# Autodesk Inventor assembly: zlozenie_wszystko
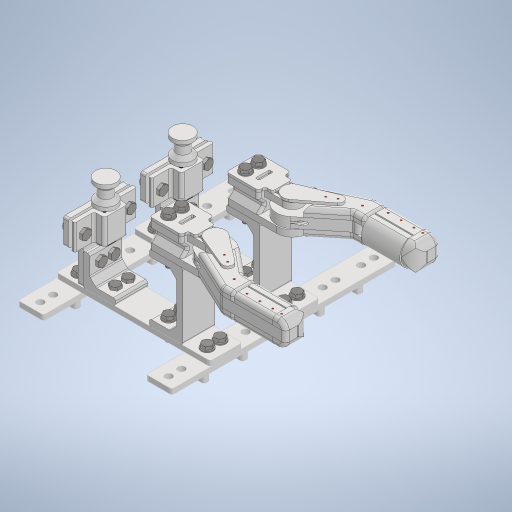
[picture p0: Inventor's stored thumbnail of the model, 512x512]
Saved by Autodesk Inventor 2024.2 (Build 282272000, 272)
## iProperties
Created: 2024-01-20
Part Number: zlozenie_wszystko
Document SubType Name: Assembly
Designer: Konrad
Author: Konrad
## Documents named in this file (9)
- D:\Inventor\magisterka\prototyp_2\zlozenie_wszystko.iam
- D:\Inventor\magisterka\prototyp_2\zlozenie_palec_lewy.iam
- D:\Inventor\magisterka\prototyp_2\zlozenie_palec_prawy.iam
- D:\Inventor\magisterka\prototyp_2\zlozenie_ramka.iam
- C:\Users\Konrad\Documents\Inventor\Content Center Files\R2024\pl-PL\DIN 125-1  A\DIN 125 - A 4,3.ipt
- C:\Users\Konrad\Documents\Inventor\Content Center Files\R2024\pl-PL\DIN EN 24 017\ISO 4017 - M4 x 16DIN EN.ipt
- C:\Users\Konrad\Documents\Inventor\Content Center Files\R2024\pl-PL\DIN 934\DIN 934 - M4 x 0,7.ipt
- D:\Inventor\magisterka\prototyp_2\zlozenie_naped_v2.iam
- C:\Users\Konrad\Documents\Inventor\Content Center Files\R2024\pl-PL\DIN 933\DIN 933 - M4  x 14.ipt
## Components (29 placed, 8 different names)
1. zlozenie_palec_lewy:1 [sub-assembly] — Zestawiające:2, Zestawiające:10, Zestawiające:11, Zestawiające:66, Równoległe:3, Zestawiające:67, Zestawiające:68, Zestawiające:69, Zestawiające:70, Zestawiające:71, Zestawiające:72, Zestawiające:74
2. zlozenie_palec_prawy:1 [sub-assembly] — Zestawiające:1, Zestawiające:9, Zestawiające:12, Zestawiające:13, Zestawiające:14, Zestawiające:15, Zestawiające:16, Zestawiające:29, Zestawiające:31
3. zlozenie_ramka:1 [sub-assembly] — Zestawiające:1, Zestawiające:2, Zestawiające:9, Zestawiające:10, Zestawiające:11, Zestawiające:12, Zestawiające:30, Zestawiające:32, Zestawiające:45, Równoległe:1, Zestawiające:46, Równoległe:2, Zestawiające:47, Zestawiające:48, Zestawiające:51, Zestawiające:53, Zestawiające:55, Zestawiające:58, Zestawiające:59, Zestawiające:60, Zestawiające:61, Zestawiające:62, Zestawiające:63, Zestawiające:64, Zestawiające:65, Zestawiające:66, Równoległe:3, Zestawiające:67, Zestawiające:73, Zestawiające:75
4. DIN 125-1 A A 4,3:1 — Zestawiające:13, Zestawiające:14, Wstawiające:1
5. DIN EN 24017 M4 x 16:1 — Wstawiające:1
6. DIN 934 - zastąpiona przez DIN EN 24032/28673/28674 M4:1 — Zestawiające:29, Zestawiające:30
7. DIN 125-1 A A 4,3:2 — Zestawiające:15, Zestawiające:16, Wstawiające:2
8. DIN EN 24017 M4 x 16:2 — Wstawiające:2
9. DIN 934 - zastąpiona przez DIN EN 24032/28673/28674 M4:2 — Zestawiające:31, Zestawiające:32
10. zlozenie_naped_v2:1 [sub-assembly] — Zestawiające:45, Równoległe:1, Zestawiające:48, Zestawiające:49, Zestawiające:50, Zestawiające:52, Zestawiające:54, Zestawiające:56, Zestawiające:57
11. zlozenie_naped_v2:2 [sub-assembly] — Zestawiające:46, Równoległe:2, Zestawiające:47
12. DIN 933 - zastąpiona przez DIN EN 24017 M4  x 14:1 — Zestawiające:49, Zestawiające:50
13. DIN 125-1 A A 4,3:9 — Zestawiające:57, Zestawiające:58, Wstawiające:9
14. DIN 934 - zastąpiona przez DIN EN 24032/28673/28674 M4:9 — Wstawiające:9
15. DIN 933 - zastąpiona przez DIN EN 24017 M4  x 14:2 — Zestawiające:51, Zestawiające:52
16. DIN 933 - zastąpiona przez DIN EN 24017 M4  x 14:3 — Zestawiające:53, Zestawiające:54
17. DIN 933 - zastąpiona przez DIN EN 24017 M4  x 14:4 — Zestawiające:55, Zestawiające:56
18. DIN 125-1 A A 4,3:10 — Zestawiające:59, Zestawiające:60, Wstawiające:10
19. DIN 125-1 A A 4,3:11 — Zestawiające:61, Zestawiające:62, Wstawiające:11
20. DIN 125-1 A A 4,3:12 — Zestawiające:63, Zestawiające:64, Wstawiające:12
21. DIN 934 - zastąpiona przez DIN EN 24032/28673/28674 M4:10 — Wstawiające:10
22. DIN 934 - zastąpiona przez DIN EN 24032/28673/28674 M4:11 — Wstawiające:11
23. DIN 934 - zastąpiona przez DIN EN 24032/28673/28674 M4:12 — Wstawiające:12
24. DIN EN 24017 M4 x 16:3 — Zestawiające:68, Zestawiające:69
25. DIN 125-1 A A 4,3:13 — Zestawiające:72, Zestawiające:73, Wstawiające:13
26. DIN 934 - zastąpiona przez DIN EN 24032/28673/28674 M4:13 — Wstawiające:13
27. DIN EN 24017 M4 x 16:4 — Zestawiające:70, Zestawiające:71
28. DIN 125-1 A A 4,3:14 — Zestawiające:74, Zestawiające:75, Wstawiające:14
29. DIN 934 - zastąpiona przez DIN EN 24032/28673/28674 M4:14 — Wstawiające:14
## Relationships (56: Mate 45, Insert 8, Flush 3)
- Zestawiające:1 [Mate]: zlozenie_palec_prawy:1 ↔ zlozenie_ramka:1
- Zestawiające:2 [Mate]: zlozenie_palec_lewy:1 ↔ zlozenie_ramka:1
- Zestawiające:9 [Mate]: zlozenie_palec_prawy:1 ↔ zlozenie_ramka:1
- Zestawiające:10 [Mate]: zlozenie_palec_lewy:1 ↔ zlozenie_ramka:1
- Zestawiające:11 [Mate]: zlozenie_palec_lewy:1 ↔ zlozenie_ramka:1
- Zestawiające:12 [Mate]: zlozenie_palec_prawy:1 ↔ zlozenie_ramka:1
- Zestawiające:13 [Mate]: zlozenie_palec_prawy:1 ↔ DIN 125-1 A A 4,3:1
- Zestawiające:14 [Mate]: zlozenie_palec_prawy:1 ↔ DIN 125-1 A A 4,3:1
- Zestawiające:15 [Mate]: zlozenie_palec_prawy:1 ↔ DIN 125-1 A A 4,3:2
- Zestawiające:16 [Mate]: zlozenie_palec_prawy:1 ↔ DIN 125-1 A A 4,3:2
- Wstawiające:1 [Insert]: DIN 125-1 A A 4,3:1 ↔ DIN EN 24017 M4 x 16:1
- Wstawiające:2 [Insert]: DIN 125-1 A A 4,3:2 ↔ DIN EN 24017 M4 x 16:2
- Zestawiające:29 [Mate]: zlozenie_palec_prawy:1 ↔ DIN 934 - zastąpiona przez DIN EN 24032/28673/28674 M4:1
- Zestawiające:30 [Mate]: zlozenie_ramka:1 ↔ DIN 934 - zastąpiona przez DIN EN 24032/28673/28674 M4:1
- Zestawiające:31 [Mate]: zlozenie_palec_prawy:1 ↔ DIN 934 - zastąpiona przez DIN EN 24032/28673/28674 M4:2
- Zestawiające:32 [Mate]: zlozenie_ramka:1 ↔ DIN 934 - zastąpiona przez DIN EN 24032/28673/28674 M4:2
- Zestawiające:45 [Mate]: zlozenie_ramka:1 ↔ zlozenie_naped_v2:1
- Równoległe:1 [Flush]: zlozenie_ramka:1 ↔ zlozenie_naped_v2:1
- Zestawiające:46 [Mate]: zlozenie_ramka:1 ↔ zlozenie_naped_v2:2
- Równoległe:2 [Flush]: zlozenie_ramka:1 ↔ zlozenie_naped_v2:2
- Zestawiające:47 [Mate]: zlozenie_ramka:1 ↔ zlozenie_naped_v2:2
- Zestawiające:48 [Mate]: zlozenie_ramka:1 ↔ zlozenie_naped_v2:1
- Zestawiające:49 [Mate]: zlozenie_naped_v2:1 ↔ DIN 933 - zastąpiona przez DIN EN 24017 M4  x 14:1
- Zestawiające:50 [Mate]: zlozenie_naped_v2:1 ↔ DIN 933 - zastąpiona przez DIN EN 24017 M4  x 14:1
- Zestawiające:51 [Mate]: zlozenie_ramka:1 ↔ DIN 933 - zastąpiona przez DIN EN 24017 M4  x 14:2
- Zestawiające:52 [Mate]: zlozenie_naped_v2:1 ↔ DIN 933 - zastąpiona przez DIN EN 24017 M4  x 14:2
- Zestawiające:53 [Mate]: zlozenie_ramka:1 ↔ DIN 933 - zastąpiona przez DIN EN 24017 M4  x 14:3
- Zestawiające:54 [Mate]: zlozenie_naped_v2:1 ↔ DIN 933 - zastąpiona przez DIN EN 24017 M4  x 14:3
- Zestawiające:55 [Mate]: zlozenie_ramka:1 ↔ DIN 933 - zastąpiona przez DIN EN 24017 M4  x 14:4
- Zestawiające:56 [Mate]: zlozenie_naped_v2:1 ↔ DIN 933 - zastąpiona przez DIN EN 24017 M4  x 14:4
- Zestawiające:57 [Mate]: zlozenie_naped_v2:1 ↔ DIN 125-1 A A 4,3:9
- Zestawiające:58 [Mate]: zlozenie_ramka:1 ↔ DIN 125-1 A A 4,3:9
- Zestawiające:59 [Mate]: zlozenie_ramka:1 ↔ DIN 125-1 A A 4,3:10
- Zestawiające:60 [Mate]: zlozenie_ramka:1 ↔ DIN 125-1 A A 4,3:10
- Zestawiające:61 [Mate]: zlozenie_ramka:1 ↔ DIN 125-1 A A 4,3:11
- Zestawiające:62 [Mate]: zlozenie_ramka:1 ↔ DIN 125-1 A A 4,3:11
- Zestawiające:63 [Mate]: zlozenie_ramka:1 ↔ DIN 125-1 A A 4,3:12
- Zestawiające:64 [Mate]: zlozenie_ramka:1 ↔ DIN 125-1 A A 4,3:12
- Wstawiające:9 [Insert]: DIN 125-1 A A 4,3:9 ↔ DIN 934 - zastąpiona przez DIN EN 24032/28673/28674 M4:9
- Wstawiające:10 [Insert]: DIN 125-1 A A 4,3:10 ↔ DIN 934 - zastąpiona przez DIN EN 24032/28673/28674 M4:10
- Wstawiające:11 [Insert]: DIN 125-1 A A 4,3:11 ↔ DIN 934 - zastąpiona przez DIN EN 24032/28673/28674 M4:11
- Wstawiające:12 [Insert]: DIN 125-1 A A 4,3:12 ↔ DIN 934 - zastąpiona przez DIN EN 24032/28673/28674 M4:12
- Zestawiające:65 [Mate]: zlozenie_ramka:1
- Zestawiające:66 [Mate]: zlozenie_palec_lewy:1 ↔ zlozenie_ramka:1
- Równoległe:3 [Flush]: zlozenie_palec_lewy:1 ↔ zlozenie_ramka:1
- Zestawiające:67 [Mate]: zlozenie_palec_lewy:1 ↔ zlozenie_ramka:1
- Zestawiające:68 [Mate]: zlozenie_palec_lewy:1 ↔ DIN EN 24017 M4 x 16:3
- Zestawiające:69 [Mate]: zlozenie_palec_lewy:1 ↔ DIN EN 24017 M4 x 16:3
- Zestawiające:70 [Mate]: zlozenie_palec_lewy:1 ↔ DIN EN 24017 M4 x 16:4
- Zestawiające:71 [Mate]: zlozenie_palec_lewy:1 ↔ DIN EN 24017 M4 x 16:4
- Zestawiające:72 [Mate]: zlozenie_palec_lewy:1 ↔ DIN 125-1 A A 4,3:13
- Zestawiające:73 [Mate]: zlozenie_ramka:1 ↔ DIN 125-1 A A 4,3:13
- Zestawiające:74 [Mate]: zlozenie_palec_lewy:1 ↔ DIN 125-1 A A 4,3:14
- Zestawiające:75 [Mate]: zlozenie_ramka:1 ↔ DIN 125-1 A A 4,3:14
- Wstawiające:13 [Insert]: DIN 125-1 A A 4,3:13 ↔ DIN 934 - zastąpiona przez DIN EN 24032/28673/28674 M4:13
- Wstawiające:14 [Insert]: DIN 125-1 A A 4,3:14 ↔ DIN 934 - zastąpiona przez DIN EN 24032/28673/28674 M4:14
